# Autodesk Inventor assembly: 全体アセンブリ２
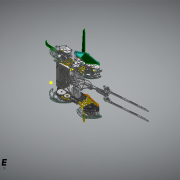
[picture p0: Inventor's stored thumbnail of the model, 180x180]
Saved by Autodesk Inventor 2020 (Build 240168000, 168)
## iProperties
Created: 2019-11-21
Part Number: 全体アセンブリ２
Material: 一般
Document SubType Name: Assembly
Designer: tanjihayato
Mass: 2720.31 g
Surface Area: 9702.1 cm^2
Volume: 1426.71 cm^3
Density: 1.90669 g/cm^3
Author: tanjihayato
## Documents named in this file (17)
- \\Mac\Home\Documents\Inventor\2019お遊び機体\全体アセンブリ２.iam
- \\Mac\Home\Documents\Inventor\2019お遊び機体\右足アセンブリ.iam
- \\Mac\Home\Documents\Inventor\2019お遊び機体\右足アセンブリ_MIR.iam
- \\Mac\Home\Documents\Inventor\2019お遊び機体\バッテリー.ipt
- \\Mac\Home\Documents\Inventor\2019お遊び機体\ウイング仮.ipt
- \\Mac\Home\Documents\Inventor\2019お遊び機体\ウイング土台.ipt
- \\Mac\Home\Documents\Inventor\2019お遊び機体\ウイング抑え.ipt
- \\Mac\Home\Documents\Inventor\2019お遊び機体\スペーサ　m3-l6.ipt
- \\Mac\Home\Documents\Inventor\2019お遊び機体\下板.ipt
- \\Mac\Home\Documents\Inventor\2019お遊び機体\バッテリーボックス.ipt
- \\Mac\Home\Documents\Inventor\2019お遊び機体\スペーサ　m3-l10.ipt
- \\Mac\Home\Documents\Inventor\2019お遊び機体\バッテリーボックス後ろ.ipt
- \\Mac\Home\Documents\Inventor\2019お遊び機体\転倒補助.ipt
- \\Mac\Home\Documents\Inventor\2019お遊び機体\後ろウイング根本.ipt
- \\Mac\Home\Documents\Inventor\2019お遊び機体\後ろウイング先端.ipt
- \\Mac\Home\Documents\Inventor\2019お遊び機体\アームアセンブリ改.iam
- \\Mac\Home\Documents\Inventor\2019お遊び機体\横回転ユニット改.iam
## Components (20 placed, 16 different names)
1. 右足アセンブリ:1 [sub-assembly] — メイト:3, メイト:5, メイト:6, 挿入:7, 挿入:9, メイト:16, 挿入:13, メイト:17
2. 右足アセンブリ_MIR:1 [sub-assembly] — メイト:3, メイト:5, メイト:6, 挿入:1, メイト:8, 挿入:10
3. バッテリー:1 — メイト:4, フラッシュ:1, フラッシュ:2
4. バッテリー:2 — メイト:4, フラッシュ:1, フラッシュ:2
5. ウイング仮:1 — メイト:9, 挿入:4
6. ウイング土台:1 — 挿入:1, メイト:8, 挿入:2, 挿入:3, メイト:9
7. ウイング抑え:1 — 挿入:5, メイト:10
8. スペーサ　m3-l6:1 — 挿入:2, メイト:10
9. スペーサ　m3-l6:2 — 挿入:3, 挿入:4, 挿入:5
10. 下板:1 — 挿入:13, メイト:17, メイト:18, メイト:19
11. バッテリーボックス:1
12. スペーサ　m3-l10:1 — 挿入:7, 挿入:8
13. バッテリーボックス:2 — 挿入:8, フラッシュ:10
14. バッテリーボックス後ろ:1 — フラッシュ:10
15. 転倒補助:1 — 挿入:10
16. 転倒補助:2 — 挿入:9, 挿入:12
17. 後ろウイング根本:1 — 挿入:11, 挿入:12, メイト:16
18. 後ろウイング先端:1 — 挿入:11
19. アームアセンブリ改:1 [sub-assembly]
20. 横回転ユニット改:1 [sub-assembly] — メイト:18, メイト:19
## Relationships (26: Insert 12, Mate 11, Flush 3)
- メイト:3 [Mate] (-320 mm): 右足アセンブリ:1 ↔ 右足アセンブリ_MIR:1
- メイト:4 [Mate]: バッテリー:1 ↔ バッテリー:2
- フラッシュ:1 [Flush]: バッテリー:1 ↔ バッテリー:2
- フラッシュ:2 [Flush]: バッテリー:1 ↔ バッテリー:2
- メイト:5 [Mate]: 右足アセンブリ:1 ↔ 右足アセンブリ_MIR:1
- メイト:6 [Mate]: 右足アセンブリ:1 ↔ 右足アセンブリ_MIR:1
- 挿入:1 [Insert]: 右足アセンブリ_MIR:1 ↔ ウイング土台:1
- メイト:8 [Mate]: 右足アセンブリ_MIR:1 ↔ ウイング土台:1
- 挿入:2 [Insert]: ウイング土台:1 ↔ スペーサ　m3-l6:1
- 挿入:3 [Insert]: ウイング土台:1 ↔ スペーサ　m3-l6:2
- メイト:9 [Mate]: ウイング仮:1 ↔ ウイング土台:1
- 挿入:4 [Insert]: ウイング仮:1 ↔ スペーサ　m3-l6:2
- 挿入:5 [Insert]: ウイング抑え:1 ↔ スペーサ　m3-l6:2
- メイト:10 [Mate]: ウイング抑え:1 ↔ スペーサ　m3-l6:1
- 挿入:7 [Insert]: 右足アセンブリ:1 ↔ スペーサ　m3-l10:1
- 挿入:8 [Insert]: スペーサ　m3-l10:1 ↔ バッテリーボックス:2
- フラッシュ:10 [Flush]: バッテリーボックス:2 ↔ バッテリーボックス後ろ:1
- 挿入:9 [Insert]: 右足アセンブリ:1 ↔ 転倒補助:2
- 挿入:10 [Insert]: 右足アセンブリ_MIR:1 ↔ 転倒補助:1
- 挿入:11 [Insert]: 後ろウイング根本:1 ↔ 後ろウイング先端:1
- 挿入:12 [Insert]: 転倒補助:2 ↔ 後ろウイング根本:1
- メイト:16 [Mate]: 右足アセンブリ:1 ↔ 後ろウイング根本:1
- 挿入:13 [Insert]: 右足アセンブリ:1 ↔ 下板:1
- メイト:17 [Mate]: 右足アセンブリ:1 ↔ 下板:1
- メイト:18 [Mate]: 下板:1 ↔ 横回転ユニット改:1
- メイト:19 [Mate]: 下板:1 ↔ 横回転ユニット改:1
